# Autodesk Inventor assembly: Chassis
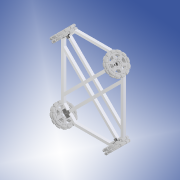
[picture p0: Inventor's stored thumbnail of the model, 180x180]
Saved by Autodesk Inventor 2017 (Build 210142000, 142)
## iProperties
Created: 2017-06-13
Part Number: Chassis
Document SubType Name: Assembly
Designer: zallen
Mass: 2624.68 g
Surface Area: 12822.9 cm^2
Volume: 1698.76 cm^3
Density: 1.54505 g/cm^3
Author: zallen
## Documents named in this file (7)
- C:\Users\zallen\Documents\GitHub\cr-laundry-robot\src\Base 2\Chassis\Chassis.iam
- C:\Users\zallen\Documents\GitHub\cr-laundry-robot\src\Base 2\Chassis\C001.ipt
- C:\Users\zallen\Documents\GitHub\cr-laundry-robot\src\Base 2\Chassis\C002.ipt
- C:\Users\zallen\Documents\GitHub\cr-laundry-robot\src\Base 2\Chassis\C003.ipt
- C:\Users\zallen\Documents\GitHub\cr-laundry-robot\src\Base 2\Chassis\C004.ipt
- C:\Users\zallen\Documents\GitHub\cr-laundry-robot\src\Base 2\Chassis\C005.ipt
- C:\Users\zallen\Documents\GitHub\cr-laundry-robot\src\Base 2\Chassis\217-2585.ipt
## Components (20 placed, 6 different names)
1. C001:1 — Mate:2, Mate:3, Mate:10, Mate:11, Mate:20, Mate:24
2. C001:2 — Mate:4, Mate:5, Mate:12, Mate:13, Mate:18, Mate:52
3. C002:1 — Mate:2, Mate:3, Mate:6, Mate:7, Mate:22, Mate:44
4. C002:2 — Mate:4, Mate:5, Mate:8, Mate:9, Mate:25, Mate:46
5. C003:1 — Mate:6, Mate:7, Mate:8, Mate:9
6. C002:3 — Mate:10, Mate:11, Mate:39, Mate:53
7. C002:4 — Mate:12, Mate:13, Mate:14, Mate:17, Mate:41, Mate:54, Mate:60, Mate:61, Mate:62
8. C003:2 — Mate:14, Mate:17, Mate:60, Mate:61, Mate:62
9. C004:1 — Mate:18, Mate:53, Mate:57, Mate:58, Mate:59
10. C004:2 — Mate:20, Mate:54, Mate:56
11. C004:3 — Mate:22, Mate:52, Mate:55
12. C004:4 — Mate:24, Mate:25, Mate:47
13. C005:1 — Mate:31, Mate:39, Mate:40, Mate:57, Mate:58
14. 217-2585:1 — Mate:31, Mate:40
15. C005:2 — Mate:41, Mate:43, Mate:56
16. 217-2585:2 — Mate:43
17. C005:3 — Mate:44, Mate:50, Mate:51, Mate:55
18. C005:4 — Mate:46, Mate:47, Mate:48, Mate:49
19. 217-2585:3 — Mate:48, Mate:49
20. 217-2585:4 — Mate:50, Mate:51
## Relationships (43: Mate 43)
- Mate:2: C001:1 ↔ C002:1
- Mate:3: C001:1 ↔ C002:1
- Mate:4: C001:2 ↔ C002:2
- Mate:5: C001:2 ↔ C002:2
- Mate:6: C002:1 ↔ C003:1
- Mate:7: C002:1 ↔ C003:1
- Mate:8: C002:2 ↔ C003:1
- Mate:9: C002:2 ↔ C003:1
- Mate:10: C001:1 ↔ C002:3
- Mate:11: C001:1 ↔ C002:3
- Mate:12: C001:2 ↔ C002:4
- Mate:13: C001:2 ↔ C002:4
- Mate:14: C002:4 ↔ C003:2
- Mate:17: C002:4 ↔ C003:2
- Mate:18: C001:2 ↔ C004:1
- Mate:20: C001:1 ↔ C004:2
- Mate:22: C002:1 ↔ C004:3
- Mate:24: C001:1 ↔ C004:4
- Mate:25: C002:2 ↔ C004:4
- Mate:31: C005:1 ↔ 217-2585:1
- [Mate]: C005:2 ↔ 217-2585:2
- Mate:39: C002:3 ↔ C005:1
- Mate:40: C005:1 ↔ 217-2585:1
- Mate:41: C002:4 ↔ C005:2
- Mate:43: C005:2 ↔ 217-2585:2
- Mate:44: C002:1 ↔ C005:3
- Mate:46: C002:2 ↔ C005:4
- Mate:47: C004:4 ↔ C005:4
- Mate:48: C005:4 ↔ 217-2585:3
- Mate:49: C005:4 ↔ 217-2585:3
- Mate:50: C005:3 ↔ 217-2585:4
- Mate:51: C005:3 ↔ 217-2585:4
- Mate:52: C001:2 ↔ C004:3
- Mate:53: C002:3 ↔ C004:1
- Mate:54: C002:4 ↔ C004:2
- Mate:55: C004:3 ↔ C005:3
- Mate:56: C004:2 ↔ C005:2
- Mate:57: C004:1 ↔ C005:1
- Mate:58: C004:1 ↔ C005:1
- Mate:59: C004:1
- Mate:60: C002:4 ↔ C003:2
- Mate:61: C002:4 ↔ C003:2
- Mate:62: C002:4 ↔ C003:2
## Named parameters: d36_d33 = 0 mm
